# Autodesk Inventor assembly: CompBot 2019
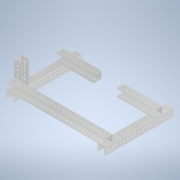
[picture p0: Inventor's stored thumbnail of the model, 180x180]
Saved by Autodesk Inventor 2020.1 (Build 241239000, 239)
## iProperties
Created: 2019-10-11
Part Number: CompBot 2019
Document SubType Name: Assembly
Designer: alpha
Author: alpha
## Documents named in this file (5)
- B:\Documents\GitHub\AO_Robotics\CAD\Projects\Joshua Schmidt\CompBot 2019.iam
- B:\Documents\GitHub\AO_Robotics\CAD\Parts Kits\FTC Tetrix KOP Organized (7-24-19)\Frame Hardware\Tetrix_39069.ipt
- B:\Documents\GitHub\AO_Robotics\CAD\Parts Kits\FTC Tetrix KOP Organized (7-24-19)\Frame Hardware\Tetrix_39068.ipt
- B:\Documents\GitHub\AO_Robotics\CAD\Parts Kits\FTC Tetrix KOP Organized (7-24-19)\Frame Hardware\Tetrix_39067.ipt
- B:\Documents\GitHub\AO_Robotics\CAD\Parts Kits\FTC Tetrix KOP Organized (7-24-19)\Frame Hardware\Tetrix_39066.ipt
## Components (6 placed, 4 different names)
1. Tetrix_39069:1 — Mate:1, Mate:2, Flush:6, Rotational:5, Flush:7, Rotational:6, Flush:8, Rotational:10
2. Tetrix_39068:1 — Flush:4, Flush:6, Rotational:5, Flush:7, Rotational:8, Flush:9
3. Tetrix_39068:2 — Flush:5, Rotational:6, Flush:8, Rotational:9
4. Tetrix_39067:2 — Flush:4, Rotational:8
5. Tetrix_39067:3 — Flush:5, Rotational:9
6. Tetrix_39066:1 — Rotational:10, Flush:9
## Relationships (13: Flush 6, RevoluteJoint 5, Mate 2)
- Mate:1: Tetrix_39069:1
- Mate:2: Tetrix_39069:1
- Flush:4: Tetrix_39068:1 ↔ Tetrix_39067:2
- Flush:5: Tetrix_39068:2 ↔ Tetrix_39067:3
- Flush:6: Tetrix_39069:1 ↔ Tetrix_39068:1
- Rotational:5 [RevoluteJoint]: Tetrix_39069:1 ↔ Tetrix_39068:1
- Flush:7: Tetrix_39069:1 ↔ Tetrix_39068:1
- Rotational:6 [RevoluteJoint]: Tetrix_39069:1 ↔ Tetrix_39068:2
- Flush:8: Tetrix_39069:1 ↔ Tetrix_39068:2
- Rotational:8 [RevoluteJoint]: Tetrix_39068:1 ↔ Tetrix_39067:2
- Rotational:9 [RevoluteJoint]: Tetrix_39068:2 ↔ Tetrix_39067:3
- Rotational:10 [RevoluteJoint]: Tetrix_39069:1 ↔ Tetrix_39066:1
- Flush:9: Tetrix_39068:1 ↔ Tetrix_39066:1
